# Autodesk Inventor assembly: restrainer
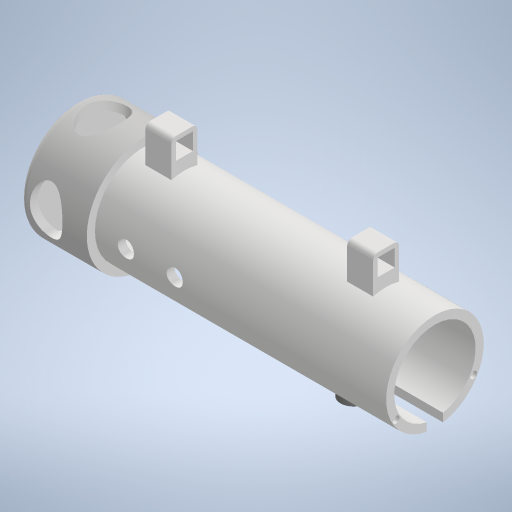
[picture p0: Inventor's stored thumbnail of the model, 512x512]
Saved by Autodesk Inventor 2023 (Build 270158000, 158)
## iProperties
Created: 2022-11-03
Part Number: restrainer
Document SubType Name: Assembly
Designer: Admin
Author: Admin
## Documents named in this file (5)
- D:\multimate\Mouse_restrainer_V3\restrainer.iam
- D:\multimate\Mouse_restrainer_V3\restrainer_middle.ipt
- D:\multimate\Mouse_restrainer_V3\restrainer_front_electrical_magnets.ipt
- D:\multimate\Mouse_restrainer_V3\restrainer_back_slider.ipt
- D:\multimate\Mouse_restrainer_V3\restrainer_back_screw.ipt
## Components (4 placed, 4 different names)
1. restrainer_middle:1 — Rotational:1, Mate:2
2. restrainer_front_electrical_magnets:1 — Rotational:1
3. restrainer_back_slider:1 — Rigid:1, Mate:2
4. restrainer_back_screw:1 — Rigid:1
## Relationships (3: RevoluteJoint 1, WeldJoint 1, Mate 1)
- Rotational:1 [RevoluteJoint] (15 mm): restrainer_middle:1 ↔ restrainer_front_electrical_magnets:1
- Rigid:1 [WeldJoint] (2.5 mm): restrainer_back_slider:1 ↔ restrainer_back_screw:1
- Mate:2: restrainer_middle:1 ↔ restrainer_back_slider:1
